# Autodesk Inventor assembly: Assembly1
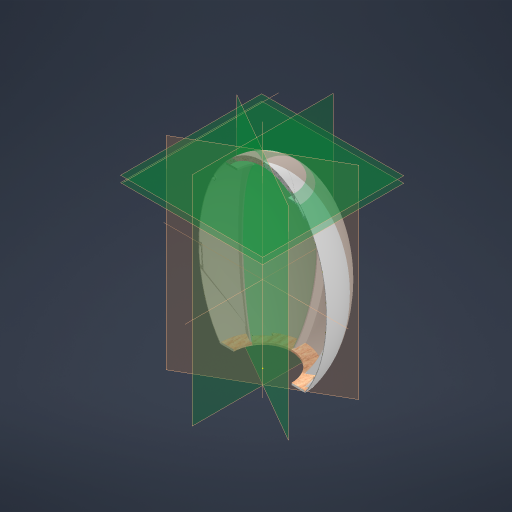
[picture p0: Inventor's stored thumbnail of the model, 512x512]
Saved by Autodesk Inventor 2023 (Build 270158000, 158)
## iProperties
Created: 2022-06-17
Part Number: Assembly1
Document SubType Name: Assembly
Designer: bananenbrot
Author: bananenbrot
## Documents named in this file (6)
- D:\fusion-zauberstab\inventor\Assembly1.iam
- D:\fusion-zauberstab\inventor\vase_v2._tom.ipt
- D:\fusion-zauberstab\inventor\Spant.ipt
- D:\fusion-zauberstab\inventor\top_centering_ring.ipt
- D:\fusion-zauberstab\inventor\lower_centering_ring.ipt
- D:\fusion-zauberstab\inventor\Spant2.ipt
## Components (9 placed, 5 different names)
1. vase_v2._tom:1 — Mate:1, Mate:2, Flush:2, Flush:3, Flush:4, Flush:5, Flush:7, Mate:3, Angle:1, Flush:8, Flush:9
2. top_centering_ring:1 — Flush:4, Flush:5
3. lower_centering_ring:1 — Flush:7
4. Spant:1 — Flush:1, Flush:3
5. Spant:2
6. Spant:3
7. Spant2:1 — Flush:8, Flush:9
8. Spant2:2
9. Spant2:3
## Component patterns: (3 elements, first: Spant:1), (3 elements, first: Spant2:1)
## Relationships (12: Flush 8, Mate 3, Angle 1)
- Mate:1: vase_v2._tom:1
- Mate:2: vase_v2._tom:1
- Flush:1: Spant:1
- Flush:2: vase_v2._tom:1
- Flush:3: vase_v2._tom:1 ↔ Spant:1
- Flush:4: vase_v2._tom:1 ↔ top_centering_ring:1
- Flush:5: vase_v2._tom:1 ↔ top_centering_ring:1
- Flush:7: vase_v2._tom:1 ↔ lower_centering_ring:1
- Mate:3: vase_v2._tom:1
- Angle:1 (45 deg): vase_v2._tom:1
- Flush:8: vase_v2._tom:1 ↔ Spant2:1
- Flush:9: vase_v2._tom:1 ↔ Spant2:1
